# Autodesk Inventor assembly: PuertaMarco
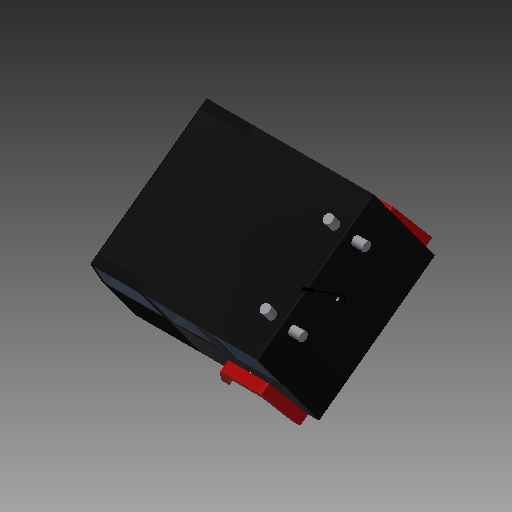
[picture p0: Inventor's stored thumbnail of the model, 512x512]
Saved by Autodesk Inventor 2017 (Build 210142000, 142)
## iProperties
Part Number: PuertaMarco
Material: Genérico
Document SubType Name: Assembly
Designer: Ghost
Author: Ghost
## Documents named in this file (8)
- C:\Users\Ghost\Desktop\UVG Semestre 8\Dibujo Mecanico\ProyectoTransformer\ProyectoTransformer\PuertaMarco.iam
- C:\Users\Ghost\Desktop\UVG Semestre 8\Dibujo Mecanico\ProyectoTransformer\ProyectoTransformer\PuertaAtras.ipt
- C:\Users\Ghost\Desktop\UVG Semestre 8\Dibujo Mecanico\ProyectoTransformer\ProyectoTransformer\Ventana.ipt
- C:\Users\Ghost\Desktop\UVG Semestre 8\Dibujo Mecanico\ProyectoTransformer\ProyectoTransformer\VentanaDelantera.ipt
- C:\Users\Ghost\Desktop\UVG Semestre 8\Dibujo Mecanico\ProyectoTransformer\ProyectoTransformer\Puerta.ipt
- C:\Users\Ghost\Desktop\UVG Semestre 8\Dibujo Mecanico\ProyectoTransformer\ProyectoTransformer\Puerta_MIR.ipt
- C:\Users\Ghost\Desktop\UVG Semestre 8\Dibujo Mecanico\ProyectoTransformer\ProyectoTransformer\VentanaLateralDelantera.ipt
- C:\Users\Ghost\Desktop\UVG Semestre 8\Dibujo Mecanico\ProyectoTransformer\ProyectoTransformer\VentanaLateralDelantera_MIR.ipt
## Components (10 placed, 7 different names)
1. PuertaAtras:1 — Coincidencia:3, Coincidencia:4, Coincidencia:5, Coincidencia:6, Coincidencia:7, Coincidencia:8, Coincidencia:9, Coincidencia:10, Coincidencia:13, Coincidencia:14, Coincidencia:15, Coincidencia:16, Coincidencia:17, Coincidencia:18, Coincidencia:23, Coincidencia:24
2. Ventana:1 — Coincidencia:5, Coincidencia:6
3. Ventana:2 — Coincidencia:3, Coincidencia:4
4. Ventana:3 — Coincidencia:7, Coincidencia:8
5. Ventana:4 — Coincidencia:9, Coincidencia:10
6. Puerta:1 — Coincidencia:14, Coincidencia:15, Coincidencia:21, Coincidencia:22
7. Puerta_MIR:1 — Coincidencia:13, Coincidencia:16, Coincidencia:17, Coincidencia:18, Coincidencia:19, Coincidencia:20
8. VentanaLateralDelantera:1 — Coincidencia:19, Coincidencia:20
9. VentanaLateralDelantera_MIR:1 — Coincidencia:21, Coincidencia:22
10. VentanaDelantera:1 — Coincidencia:23, Coincidencia:24
## Relationships (20: Mate 20)
- Coincidencia:3 [Mate]: PuertaAtras:1 ↔ Ventana:2
- Coincidencia:4 [Mate]: PuertaAtras:1 ↔ Ventana:2
- Coincidencia:5 [Mate]: PuertaAtras:1 ↔ Ventana:1
- Coincidencia:6 [Mate]: PuertaAtras:1 ↔ Ventana:1
- Coincidencia:7 [Mate]: PuertaAtras:1 ↔ Ventana:3
- Coincidencia:8 [Mate]: PuertaAtras:1 ↔ Ventana:3
- Coincidencia:9 [Mate]: PuertaAtras:1 ↔ Ventana:4
- Coincidencia:10 [Mate]: PuertaAtras:1 ↔ Ventana:4
- Coincidencia:13 [Mate]: PuertaAtras:1 ↔ Puerta_MIR:1
- Coincidencia:14 [Mate]: PuertaAtras:1 ↔ Puerta:1
- Coincidencia:15 [Mate]: PuertaAtras:1 ↔ Puerta:1
- Coincidencia:16 [Mate]: PuertaAtras:1 ↔ Puerta_MIR:1
- Coincidencia:17 [Mate]: PuertaAtras:1 ↔ Puerta_MIR:1
- Coincidencia:18 [Mate]: PuertaAtras:1 ↔ Puerta_MIR:1
- Coincidencia:19 [Mate]: Puerta_MIR:1 ↔ VentanaLateralDelantera:1
- Coincidencia:20 [Mate]: Puerta_MIR:1 ↔ VentanaLateralDelantera:1
- Coincidencia:21 [Mate]: Puerta:1 ↔ VentanaLateralDelantera_MIR:1
- Coincidencia:22 [Mate]: Puerta:1 ↔ VentanaLateralDelantera_MIR:1
- Coincidencia:23 [Mate]: PuertaAtras:1 ↔ VentanaDelantera:1
- Coincidencia:24 [Mate]: PuertaAtras:1 ↔ VentanaDelantera:1
